# Autodesk Inventor assembly: Note
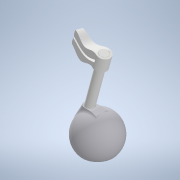
[picture p0: Inventor's stored thumbnail of the model, 180x180]
Saved by Autodesk Inventor 2020 (Build 240168000, 168)
## iProperties
Created: 2020-05-10
Part Number: Note
Document SubType Name: Assembly
Designer: MartinDJay
Author: MartinDJay
## Documents named in this file (4)
- C:\Users\MartinDJay\Documents\GitHub\CAD_Elements\CAD\Note.iam
- C:\Users\MartinDJay\Documents\GitHub\CAD_Elements\CAD\Note.ipt
- C:\Users\MartinDJay\Documents\GitHub\CAD_Elements\CAD\Stiel.ipt
- C:\Users\MartinDJay\Documents\GitHub\CAD_Elements\CAD\Fahne.ipt
## Components (3 placed, 3 different names)
1. Note:1 — Fluchtend:1, Fluchtend:2, Fluchtend:3, Passend:1, Passend:2
2. Stiel:1 — Passend:1, Passend:2, Passend:3, Fluchtend:4
3. Fahne:1 — Passend:3, Fluchtend:4
## Relationships (7: Flush 4, Mate 3)
- Fluchtend:1 [Flush]: Note:1
- Fluchtend:2 [Flush]: Note:1
- Fluchtend:3 [Flush]: Note:1
- Passend:1 [Mate]: Note:1 ↔ Stiel:1
- Passend:2 [Mate] (-20 mm): Note:1 ↔ Stiel:1
- Passend:3 [Mate]: Stiel:1 ↔ Fahne:1
- Fluchtend:4 [Flush]: Stiel:1 ↔ Fahne:1
